# Autodesk Inventor assembly: MagnetMount
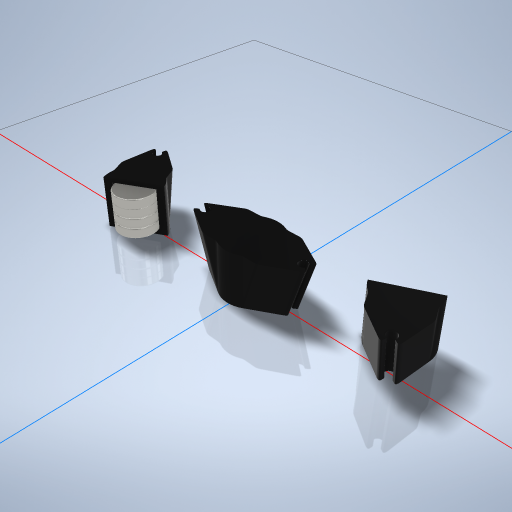
[picture p0: Inventor's stored thumbnail of the model, 512x512]
Saved by Autodesk Inventor 2023 (Build 270158000, 158)
## iProperties
Created: 2023-05-09
Part Number: MagnetMount
Document SubType Name: Assembly
Designer: Joshua
Author: Joshua
## Documents named in this file (4)
- D:\Creative Stuffs\Autodesk\BikeOdometer\MagnetMount.iam
- D:\Creative Stuffs\Autodesk\BikeOdometer\MagnetMount.ipt
- D:\Creative Stuffs\Autodesk\BikeOdometer\Cut_MagnetMount.ipt
- D:\Creative Stuffs\Autodesk\BikeOdometer\Magnet.ipt
## Components (7 placed, 3 different names)
1. MagnetMount:1
2. Cut_MagnetMount:1 — Insert:1
3. Cut_MagnetMount:2
4. Magnet:1 — Insert:4
5. Magnet:2 — Insert:1, Insert:2
6. Magnet:3 — Insert:2, Insert:3
7. Magnet:4 — Insert:3, Insert:4
## Relationships (4: Insert 4)
- Insert:1: Cut_MagnetMount:1 ↔ Magnet:2
- Insert:2: Magnet:2 ↔ Magnet:3
- Insert:3: Magnet:3 ↔ Magnet:4
- Insert:4: Magnet:1 ↔ Magnet:4
